# Autodesk Inventor assembly: Zespol1
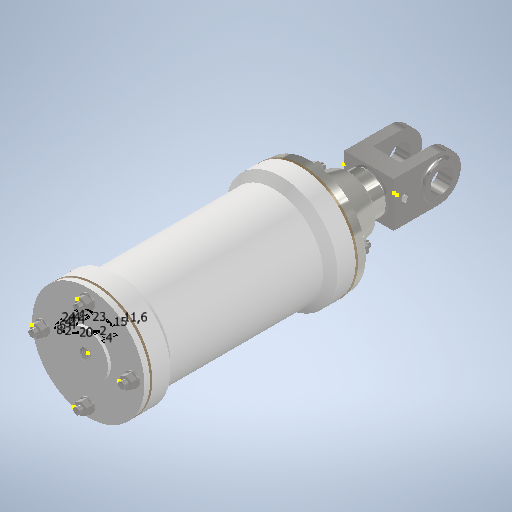
[picture p0: Inventor's stored thumbnail of the model, 512x512]
Saved by Autodesk Inventor 2025.2 (Build 292293000, 293)
## iProperties
Created: 2025-03-23
Part Number: Zespol1
Document SubType Name: Assembly
Designer: marci
Author: marci
## Documents named in this file (12)
- D:\Inventor\Podstawy_Konstrukcji_Maszyn\Projekt1_temat21\Zespol1.iam
- D:\Inventor\Podstawy_Konstrukcji_Maszyn\Projekt1_temat21\01cylinder (2).ipt
- D:\Inventor\Podstawy_Konstrukcji_Maszyn\Projekt1_temat21\02pokrywa.ipt
- D:\Inventor\Podstawy_Konstrukcji_Maszyn\Projekt1_temat21\04tloczysko.ipt
- D:\Inventor\Podstawy_Konstrukcji_Maszyn\Projekt1_temat21\7Tłok.ipt
- D:\Inventor\Podstawy_Konstrukcji_Maszyn\Projekt1_temat21\08pokrywa (2).ipt
- D:\Inventor\Podstawy_Konstrukcji_Maszyn\Projekt1_temat21\06widelki.ipt
- D:\Inventor\Podstawy_Konstrukcji_Maszyn\Projekt1_temat21\Sprężyna naciskowa11.ipt
- D:\Inventor\Podstawy_Konstrukcji_Maszyn\Projekt1_temat21\uszczelka.ipt
- D:\Inventor\Podstawy_Konstrukcji_Maszyn\Projekt1_temat21\pierśnień.ipt
- D:\Inventor\Podstawy_Konstrukcji_Maszyn\Projekt1_temat21\śróbki1.ipt
- D:\Inventor\Podstawy_Konstrukcji_Maszyn\Projekt1_temat21\kołek.ipt
## Components (20 placed, 11 different names)
1. 01cylinder (2):1 — Obrotowe:4, Obrotowe:5, Obrotowe:6, Obrotowe:7
2. 02pokrywa:1 — Obrotowe:8, Obrotowe:9, Obrotowe:10, Obrotowe:11, Obrotowe:12
3. 7Tłok:1 — Obrotowe:1, Równoległe:1, Obrotowe:2, Obrotowe:3, Obrotowe:4
4. 08pokrywa (2):1 — Obrotowe:7, Obrotowe:13, Obrotowe:14, Obrotowe:15, Obrotowe:16, Obrotowe:17
5. 06widelki:1 — Obrotowe:17, Obrotowe:18
6. 04tloczysko:1 — Obrotowe:1, Zestawiające:1
7. Sprężyna naciskowa1:2 — Zestawiające:1, Równoległe:1
8. uszczelka:1 — Obrotowe:6, Obrotowe:8
9. uszczelka:2 — Obrotowe:5
10. pierśnień:1 — Obrotowe:2
11. pierśnień:2 — Obrotowe:3
12. śróbki1:2 — Obrotowe:12
13. śróbki1:3 — Obrotowe:9
14. śróbki1:4 — Obrotowe:16
15. śróbki1:5 — Obrotowe:11
16. śróbki1:6 — Obrotowe:13
17. śróbki1:7 — Obrotowe:14
18. śróbki1:8 — Obrotowe:15
19. śróbki1:9 — Obrotowe:10
20. kołek:1 — Obrotowe:18
## Relationships (20: RevoluteJoint 18, Mate 1, Flush 1)
- Obrotowe:1 [RevoluteJoint]: 7Tłok:1 ↔ 04tloczysko:1
- Zestawiające:1 [Mate]: 04tloczysko:1 ↔ Sprężyna naciskowa1:2
- Równoległe:1 [Flush]: 7Tłok:1 ↔ Sprężyna naciskowa1:2
- Obrotowe:2 [RevoluteJoint]: 7Tłok:1 ↔ pierśnień:1
- Obrotowe:3 [RevoluteJoint]: 7Tłok:1 ↔ pierśnień:2
- Obrotowe:4 [RevoluteJoint]: 01cylinder (2):1 ↔ 7Tłok:1
- Obrotowe:5 [RevoluteJoint]: 01cylinder (2):1 ↔ uszczelka:2
- Obrotowe:6 [RevoluteJoint]: 01cylinder (2):1 ↔ uszczelka:1
- Obrotowe:7 [RevoluteJoint]: 01cylinder (2):1 ↔ 08pokrywa (2):1
- Obrotowe:8 [RevoluteJoint]: 02pokrywa:1 ↔ uszczelka:1
- Obrotowe:9 [RevoluteJoint]: 02pokrywa:1 ↔ śróbki1:3
- Obrotowe:10 [RevoluteJoint]: 02pokrywa:1 ↔ śróbki1:9
- Obrotowe:11 [RevoluteJoint]: 02pokrywa:1 ↔ śróbki1:5
- Obrotowe:12 [RevoluteJoint]: 02pokrywa:1 ↔ śróbki1:2
- Obrotowe:13 [RevoluteJoint]: 08pokrywa (2):1 ↔ śróbki1:6
- Obrotowe:14 [RevoluteJoint]: 08pokrywa (2):1 ↔ śróbki1:7
- Obrotowe:15 [RevoluteJoint]: 08pokrywa (2):1 ↔ śróbki1:8
- Obrotowe:16 [RevoluteJoint]: 08pokrywa (2):1 ↔ śróbki1:4
- Obrotowe:17 [RevoluteJoint]: 08pokrywa (2):1 ↔ 06widelki:1
- Obrotowe:18 [RevoluteJoint]: 06widelki:1 ↔ kołek:1
